# Autodesk Inventor assembly: HbIndexFinger01
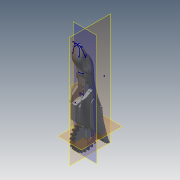
[picture p0: Inventor's stored thumbnail of the model, 180x180]
Saved by Autodesk Inventor 2015 SP1 (Build 190203100, 203)
## iProperties
Created: 2015-04-11
Part Number: HbIndexFinger01
Document SubType Name: Assembly
Designer: Yamaura
Author: Yamaura
## Documents named in this file (11)
- C:\Users\Yamaura\Documents\GitHub\HACKberry\HACKberry-hardware\3D\Inventor\Parts\HbIndexFinger01.iam
- C:\Users\Yamaura\Documents\GitHub\HACKberry\HACKberry-hardware\3D\Inventor\Parts\HbIndexInputLink02.ipt
- C:\Users\Yamaura\Documents\GitHub\HACKberry\HACKberry-hardware\3D\Inventor\Parts\TOS 0.5-6-270-5.ipt
- C:\Users\Yamaura\Documents\GitHub\HACKberry\HACKberry-hardware\3D\Inventor\Parts\HbReleaseLever01.ipt
- C:\Users\Yamaura\Documents\GitHub\HACKberry\HACKberry-hardware\3D\Inventor\Parts\HbIndexCouplerLink02.ipt
- C:\Users\Yamaura\Documents\GitHub\HACKberry\HACKberry-hardware\3D\Inventor\Parts\HbIndexCouplerLinkCover02.ipt
- C:\Users\Yamaura\Documents\GitHub\HACKberry\HACKberry-hardware\3D\Inventor\Parts\HbIndexProximalPhalanxCover02.ipt
- C:\Users\Yamaura\Documents\GitHub\HACKberry\HACKberry-hardware\3D\Inventor\Parts\HbReleaseLever02.ipt
- C:\Users\Yamaura\Documents\GitHub\HACKberry\HACKberry-hardware\3D\Inventor\Parts\HbIndexProximalPhalanx03.ipt
- C:\Users\Yamaura\Documents\GitHub\HACKberry\HACKberry-hardware\3D\Inventor\Parts\HbIndexMiddle-DistalPhalanx02.ipt
- C:\Users\Yamaura\Documents\GitHub\HACKberry\HACKberry-hardware\3D\Inventor\Parts\ScrewM2L10.ipt
## Components (15 placed, 12 different names)
1. HbIndexInputLink02_1
2. TOS 0.5-6-270-5_1
3. TOS 0.5-6-270-5_2
4. HbReleaseLever01_1
5. HbReleaseLever01_2
6. HbIndexCouplerLink02_1
7. HbIndexCouplerLinkCover02_1 — メイト:5, メイト:6, メイト:7, メイト:8
8. HbIndexProximalPhalanxCover02_1
9. HbReleaseLever02_1
10. HbIndexProximalPhalanx03_1 — メイト:1, メイト:2, メイト:3, メイト:4
11. HbIndexMiddle-DistalPhalanx02_1
12. ScrewM2L10:1 — メイト:5, メイト:6
13. ScrewM2L10:2 — メイト:7, メイト:8
14. ScrewM2L10:3 — メイト:3, メイト:4
15. ScrewM2L10:4 — メイト:1, メイト:2
## Relationships (8: Mate 8)
- メイト:1 [Mate]: HbIndexProximalPhalanx03_1 ↔ ScrewM2L10:4
- メイト:2 [Mate]: HbIndexProximalPhalanx03_1 ↔ ScrewM2L10:4
- メイト:3 [Mate]: HbIndexProximalPhalanx03_1 ↔ ScrewM2L10:3
- メイト:4 [Mate]: HbIndexProximalPhalanx03_1 ↔ ScrewM2L10:3
- メイト:5 [Mate]: HbIndexCouplerLinkCover02_1 ↔ ScrewM2L10:1
- メイト:6 [Mate]: HbIndexCouplerLinkCover02_1 ↔ ScrewM2L10:1
- メイト:7 [Mate]: HbIndexCouplerLinkCover02_1 ↔ ScrewM2L10:2
- メイト:8 [Mate]: HbIndexCouplerLinkCover02_1 ↔ ScrewM2L10:2
